# Autodesk Inventor assembly: Birdhouse Assembly 2
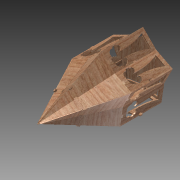
[picture p0: Inventor's stored thumbnail of the model, 180x180]
Saved by Autodesk Inventor 2015 (Build 190159000, 159)
## iProperties
Created: 2018-03-08
Part Number: Birdhouse Assembly 2
Document SubType Name: Assembly
Designer: Administrator
Author: Administrator
## Documents named in this file (7)
- L:\IED 9th\Birdhouse Assembly 2.iam
- L:\IED 9th\Star Side Out.ipt
- L:\IED 9th\Star Side.ipt
- L:\IED 9th\Star Base.ipt
- L:\IED 9th\Birdhouse Wall.ipt
- L:\IED 9th\Birdhouse Wall 2.ipt
- L:\IED 9th\Birdhouse Tree Wall.ipt
## Components (21 placed, 6 different names)
1. Star Side Out:1 — Mate:25, Mate:26, Mate:45
2. Star Side Out:2 — Mate:13, Mate:17, Mate:48
3. Star Side Out:3 — Mate:21, Mate:42
4. Star Side Out:4 — Mate:50, Mate:51
5. Star Side Out:5 — Mate:31, Mate:39
6. Star Side:1 — Mate:15, Mate:16, Mate:48
7. Star Side:2 — Mate:28, Mate:29, Mate:45
8. Star Side:3 — Mate:18, Mate:22
9. Star Side:4 — Mate:32, Mate:33
10. Star Side:5 — Mate:6, Mate:10
11. Star Base:1 — Mate:34, Mate:36, Mate:37, Mate:38, Mate:40, Mate:41, Mate:43, Mate:44, Mate:46, Mate:47, Mate:52
12. Birdhouse Wall:2 — Mate:28, Mate:29, Flush:4, Mate:46
13. Birdhouse Wall:4 — Mate:15, Mate:16, Mate:34, Flush:2, Mate:47
14. Birdhouse Wall:8 — Mate:6, Mate:10, Mate:36, Flush:1, Flush:5, Mate:37
15. Birdhouse Wall:9 — Mate:18, Mate:22, Mate:41
16. Birdhouse Wall 2:1 — Mate:25, Mate:26, Flush:3, Mate:44
17. Birdhouse Wall 2:3 — Mate:31, Mate:39, Mate:40
18. Birdhouse Wall 2:4 — Mate:21, Mate:42, Mate:43
19. Birdhouse Wall 2:5 — Mate:13, Mate:17, Flush:1, Flush:2, Flush:3, Flush:4, Mate:38
20. Birdhouse Tree Wall:1 — Mate:32, Mate:33, Flush:5
21. Birdhouse Wall 2:6 — Mate:50, Mate:51, Mate:52
## Relationships (38: Mate 33, Flush 5)
- Mate:6: Star Side:5 ↔ Birdhouse Wall:8
- Mate:10: Star Side:5 ↔ Birdhouse Wall:8
- Mate:13: Star Side Out:2 ↔ Birdhouse Wall 2:5
- Mate:15: Star Side:1 ↔ Birdhouse Wall:4
- Mate:16: Star Side:1 ↔ Birdhouse Wall:4
- Mate:17: Star Side Out:2 ↔ Birdhouse Wall 2:5
- Mate:18: Star Side:3 ↔ Birdhouse Wall:9
- Mate:21: Star Side Out:3 ↔ Birdhouse Wall 2:4
- Mate:22: Star Side:3 ↔ Birdhouse Wall:9
- Mate:25: Star Side Out:1 ↔ Birdhouse Wall 2:1
- Mate:26: Star Side Out:1 ↔ Birdhouse Wall 2:1
- Mate:28: Star Side:2 ↔ Birdhouse Wall:2
- Mate:29: Star Side:2 ↔ Birdhouse Wall:2
- Mate:31: Star Side Out:5 ↔ Birdhouse Wall 2:3
- Mate:32: Star Side:4 ↔ Birdhouse Tree Wall:1
- Mate:33: Star Side:4 ↔ Birdhouse Tree Wall:1
- Mate:34: Star Base:1 ↔ Birdhouse Wall:4
- Mate:36: Star Base:1 ↔ Birdhouse Wall:8
- Flush:1: Birdhouse Wall:8 ↔ Birdhouse Wall 2:5
- Flush:2: Birdhouse Wall:4 ↔ Birdhouse Wall 2:5
- Flush:3: Birdhouse Wall 2:1 ↔ Birdhouse Wall 2:5
- Flush:4: Birdhouse Wall:2 ↔ Birdhouse Wall 2:5
- Flush:5: Birdhouse Wall:8 ↔ Birdhouse Tree Wall:1
- Mate:37: Star Base:1 ↔ Birdhouse Wall:8
- Mate:38: Star Base:1 ↔ Birdhouse Wall 2:5
- Mate:39: Star Side Out:5 ↔ Birdhouse Wall 2:3
- Mate:40: Star Base:1 ↔ Birdhouse Wall 2:3
- Mate:41: Star Base:1 ↔ Birdhouse Wall:9
- Mate:42: Star Side Out:3 ↔ Birdhouse Wall 2:4
- Mate:43: Star Base:1 ↔ Birdhouse Wall 2:4
- Mate:44: Star Base:1 ↔ Birdhouse Wall 2:1
- Mate:45: Star Side Out:1 ↔ Star Side:2
- Mate:46: Star Base:1 ↔ Birdhouse Wall:2
- Mate:47: Star Base:1 ↔ Birdhouse Wall:4
- Mate:48: Star Side Out:2 ↔ Star Side:1
- Mate:50: Star Side Out:4 ↔ Birdhouse Wall 2:6
- Mate:51: Star Side Out:4 ↔ Birdhouse Wall 2:6
- Mate:52: Star Base:1 ↔ Birdhouse Wall 2:6
